# Autodesk Inventor assembly: AX12_XL320_Example_Assembly
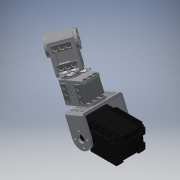
[picture p0: Inventor's stored thumbnail of the model, 180x180]
Saved by Autodesk Inventor 2017 (Build 210142000, 142)
## iProperties
Created: 2016-09-05
Part Number: AX12_XL320_Example_Assembly
Document SubType Name: Assembly
Designer: Labtech
Author: Labtech
## Documents named in this file (9)
- C:\Users\Labtech\Google Drive\OLLO Pieces\ROB550_CAD_Lib\AX12_XL320_Example_Assembly.iam
- C:\Users\Labtech\Google Drive\OLLO Pieces\ROB550_CAD_Lib\AX12.ipt
- C:\Users\Labtech\Google Drive\OLLO Pieces\ROB550_CAD_Lib\AX12_Hub.ipt
- C:\Users\Labtech\Google Drive\OLLO Pieces\ROB550_CAD_Lib\OlloToAX12.ipt
- C:\Users\Labtech\Google Drive\OLLO Pieces\ROB550_CAD_Lib\AX12_Idler.ipt
- C:\Users\Labtech\Google Drive\OLLO Pieces\ROB550_CAD_Lib\XL320.ipt
- C:\Users\Labtech\Google Drive\OLLO Pieces\ROB550_CAD_Lib\XL320_HubToOllo.ipt
- C:\Users\Labtech\Google Drive\OLLO Pieces\ROB550_CAD_Lib\XL320_HubToXL320_Base.ipt
- C:\Users\Labtech\Google Drive\OLLO Pieces\ROB550_CAD_Lib\XL320_IdlerToOllo.ipt
## Components (10 placed, 8 different names)
1. AX12:1 — Flush:1, Rotational:2
2. AX12_Hub:1 — Insert:2, Insert:3, Rotational:2
3. OlloToAX12:1 — Insert:2, Insert:3, Insert:4, Insert:5
4. AX12_Idler:1 — Flush:1
5. XL320:1 — Insert:4, Insert:5, Rotational:3
6. XL320_HubToOllo:1 — Insert:7, Insert:8, Rotational:3
7. XL320_HubToXL320_Base:1 — Insert:7, Insert:8, Insert:9, Insert:10
8. XL320:2 — Insert:9, Insert:10, Rotational:1, Insert:11
9. XL320_HubToOllo:2 — Rotational:1
10. XL320_IdlerToOllo:1 — Insert:11
## Relationships (13: Insert 9, RevoluteJoint 3, Flush 1)
- Insert:2: AX12_Hub:1 ↔ OlloToAX12:1
- Insert:3: AX12_Hub:1 ↔ OlloToAX12:1
- Flush:1: AX12:1 ↔ AX12_Idler:1
- Insert:4: OlloToAX12:1 ↔ XL320:1
- Insert:5: OlloToAX12:1 ↔ XL320:1
- Insert:7: XL320_HubToOllo:1 ↔ XL320_HubToXL320_Base:1
- Insert:8: XL320_HubToOllo:1 ↔ XL320_HubToXL320_Base:1
- Insert:9: XL320_HubToXL320_Base:1 ↔ XL320:2
- Insert:10: XL320_HubToXL320_Base:1 ↔ XL320:2
- Rotational:1 [RevoluteJoint]: XL320:2 ↔ XL320_HubToOllo:2
- Insert:11: XL320:2 ↔ XL320_IdlerToOllo:1
- Rotational:2 [RevoluteJoint]: AX12:1 ↔ AX12_Hub:1
- Rotational:3 [RevoluteJoint]: XL320:1 ↔ XL320_HubToOllo:1
